# Autodesk Inventor assembly: CP675 Fixing
Saved by Autodesk Inventor 2015 (Build 190159000, 159)
## iProperties
Created: 2014-04-07
Part Number: CP675 Fixing
Document SubType Name: Assembly
Designer: alid
Author: alid
## Documents named in this file (4)
- C:\Vault Workspace\Inventor2015new\Projects\7_Electrical\ABB\CP675\CP675 Fixing.iam
- C:\Vault Workspace\Inventor2015new\Projects\7_Electrical\ABB\CP675\ABB_CP675_Panel_Block.ipt
- C:\Vault Workspace\Inventor2015new\Projects\7_Electrical\ABB\CP675\ABB_CP675_Panel_Screw.ipt
- C:\Vault Workspace\Inventor2015new\Projects\7_Electrical\ABB\CP675\ABB_CP675_Panel_Bracket.ipt
## Components (3 placed, 3 different names)
1. ABB_CP675_Panel_Block:1
2. ABB_CP675_Panel_Screw:1
3. ABB_CP675_Panel_Bracket:1
## Relationships (2: WeldJoint 1, RevoluteJoint 1)
- [WeldJoint]: ABB_CP675_Panel_Block:1 ↔ ABB_CP675_Panel_Screw:1
- [RevoluteJoint]: ABB_CP675_Panel_Screw:1 ↔ ABB_CP675_Panel_Bracket:1
